# Autodesk Inventor assembly: Final 3D model
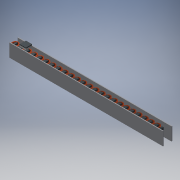
[picture p0: Inventor's stored thumbnail of the model, 180x180]
Saved by Autodesk Inventor 2019 (Build 230136000, 136)
## iProperties
Created: 2021-07-19
Part Number: Final 3D model
Document SubType Name: Assembly
Designer: pensun
Author: pensun
## Documents named in this file (6)
- C:\Pengpeng\02 coreWithCoil(Ecore)\Hyperloop\Final 3D model.iam
- C:\Pengpeng\02 coreWithCoil(Ecore)\Hyperloop\Track\plastic wall.ipt
- C:\Pengpeng\02 coreWithCoil(Ecore)\Hyperloop\Track\Final E core.iam
- C:\Pengpeng\02 coreWithCoil(Ecore)\Hyperloop\plate\al.ipt
- C:\Pengpeng\02 coreWithCoil(Ecore)\Hyperloop\plate\Iron.ipt
- C:\Pengpeng\02 coreWithCoil(Ecore)\Hyperloop\Coil\coil.ipt
## Components (29 placed, 5 different names)
1. plastic wall:1 — Mate:1, Flush:1, Mate:3, Flush:3, Mate:6
2. plastic wall:2 — Mate:1, Flush:1, Flush:2, Flush:3, Flush:4
3. Final E core:1 [sub-assembly] — Flush:2, Mate:3, Flush:4, Mate:5, Mate:7
4. al:1 — Mate:4, Flush:5, Flush:6, Mate:5, Mate:6
5. Iron:1 — Mate:4, Flush:5, Flush:6
6. coil:1 — Mate:7
7. coil:2
8. coil:3
9. coil:4
10. coil:5
11. coil:6
12. coil:7
13. coil:8
14. coil:9
15. coil:10
16. coil:11
17. coil:12
18. coil:13
19. coil:14
20. coil:15
21. coil:16
22. coil:17
23. coil:18
24. coil:19
25. coil:20
26. coil:21
27. coil:22
28. coil:23
29. coil:24
## Component patterns: (24 elements, first: coil:1)
## Relationships (12: Mate 6, Flush 6)
- Mate:1 (50 mm): plastic wall:1 ↔ plastic wall:2
- Flush:1: plastic wall:1 ↔ plastic wall:2
- Flush:2 (4 mm): plastic wall:2 ↔ Final E core:1
- Mate:3 (15 mm): plastic wall:1 ↔ Final E core:1
- Flush:3: plastic wall:1 ↔ plastic wall:2
- Flush:4: plastic wall:2 ↔ Final E core:1
- Mate:4: al:1 ↔ Iron:1
- Flush:5: al:1 ↔ Iron:1
- Flush:6: al:1 ↔ Iron:1
- Mate:5 (15 mm): Final E core:1 ↔ al:1
- Mate:6 (5 mm): plastic wall:1 ↔ al:1
- Mate:7: Final E core:1 ↔ coil:1
